# Autodesk Inventor assembly: Factions_Council
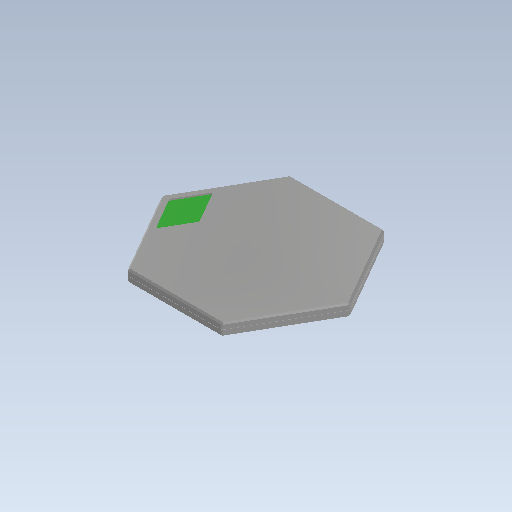
[picture p0: Inventor's stored thumbnail of the model, 512x512]
Saved by Autodesk Inventor 2021 (Build 250183000, 183)
## iProperties
Created: 2023-03-16
Part Number: Factions_Council
Document SubType Name: Assembly
Designer: Bradley
Author: Bradley
## Documents named in this file (7)
- C:\Users\Bradley\Git\TI4\Factions\Factions_Council.iam
- C:\Users\Bradley\Git\TI4\Factions\Factions_Lid.ipt
- C:\Users\Bradley\Git\TI4\Components\FactionSpecial_Council_Cards_All.ipt
- C:\Users\Bradley\Git\TI4\Components\FactionSpecial_Council_ControlMarker_Single.ipt
- C:\Users\Bradley\Git\TI4\Components\FactionSpecial_Council_Home.ipt
- C:\Users\Bradley\Git\TI4\Factions\Factions_BaseCouncil.ipt
- C:\Users\Bradley\Git\TI4\Components\FactionSpecial_Council_CommandToken_Single.ipt
## Components (38 placed, 6 different names)
1. Factions_BaseCouncil:1 — Mate:1, Mate:3, Mate:4, Mate:5, Mate:8, Mate:9, Mate:10, Mate:21, Mate:22, Mate:23, Mate:24, Mate:25, Mate:26, Mate:27, Mate:28, Mate:29, Mate:30, Mate:32, Mate:33, Mate:35, Mate:36, Mate:37, Mate:38, Mate:39, Mate:40, Mate:41, Mate:52, Mate:53, Mate:54, Mate:55, Mate:56, Mate:57, Mate:58, Mate:60, Mate:61, Mate:63, Mate:65, Flush:47, Flush:48
2. Factions_Lid:1 — Mate:1, Flush:47, Flush:48
3. FactionSpecial_Council_Cards_All:1 — Mate:3, Mate:4, Mate:5
4. FactionSpecial_Council_CommandToken_Single:1 — Mate:42, Flush:27, Flush:29, Mate:52, Mate:57, Mate:58, Mate:59
5. FactionSpecial_Council_CommandToken_Single:10
6. FactionSpecial_Council_CommandToken_Single:11 — Mate:55, Mate:63, Mate:64, Mate:66
7. FactionSpecial_Council_CommandToken_Single:12
8. FactionSpecial_Council_CommandToken_Single:13
9. FactionSpecial_Council_CommandToken_Single:14 — Mate:56, Mate:65, Mate:66
10. FactionSpecial_Council_CommandToken_Single:15
11. FactionSpecial_Council_CommandToken_Single:16
12. FactionSpecial_Council_CommandToken_Single:2 — Mate:42, Mate:43, Flush:27, Flush:28, Flush:29, Flush:30
13. FactionSpecial_Council_CommandToken_Single:3 — Mate:43, Flush:28, Flush:30
14. FactionSpecial_Council_CommandToken_Single:4 — Mate:39, Mate:40, Mate:41
15. FactionSpecial_Council_CommandToken_Single:5 — Mate:53, Mate:59, Mate:60, Mate:62
16. FactionSpecial_Council_CommandToken_Single:6
17. FactionSpecial_Council_CommandToken_Single:7
18. FactionSpecial_Council_CommandToken_Single:8 — Mate:54, Mate:61, Mate:62, Mate:64
19. FactionSpecial_Council_CommandToken_Single:9
20. FactionSpecial_Council_ControlMarker_Single:1 — Mate:6, Flush:4, Flush:5, Mate:8, Mate:9, Mate:10
21. FactionSpecial_Council_ControlMarker_Single:10 — Mate:23, Mate:30, Mate:31
22. FactionSpecial_Council_ControlMarker_Single:11
23. FactionSpecial_Council_ControlMarker_Single:12
24. FactionSpecial_Council_ControlMarker_Single:13 — Mate:24, Mate:28, Mate:29, Mate:31
25. FactionSpecial_Council_ControlMarker_Single:14
26. FactionSpecial_Council_ControlMarker_Single:15
27. FactionSpecial_Council_ControlMarker_Single:16 — Mate:25, Mate:26, Mate:27
28. FactionSpecial_Council_ControlMarker_Single:17
29. FactionSpecial_Council_ControlMarker_Single:18
30. FactionSpecial_Council_ControlMarker_Single:2 — Mate:6, Mate:7, Flush:3, Flush:4, Flush:5, Flush:6
31. FactionSpecial_Council_ControlMarker_Single:3 — Mate:7, Flush:3, Flush:6
32. FactionSpecial_Council_ControlMarker_Single:4 — Mate:21, Mate:34, Mate:35
33. FactionSpecial_Council_ControlMarker_Single:5
34. FactionSpecial_Council_ControlMarker_Single:6
35. FactionSpecial_Council_ControlMarker_Single:7 — Mate:22, Mate:32, Mate:33, Mate:34
36. FactionSpecial_Council_ControlMarker_Single:8
37. FactionSpecial_Council_ControlMarker_Single:9
38. FactionSpecial_Council_Home:1 — Mate:36, Mate:37, Mate:38
## Relationships (111: Mate 65, Flush 46)
- Mate:1: Factions_BaseCouncil:1 ↔ Factions_Lid:1
- Mate:3: Factions_BaseCouncil:1 ↔ FactionSpecial_Council_Cards_All:1
- Mate:4 (0.5 mm): Factions_BaseCouncil:1 ↔ FactionSpecial_Council_Cards_All:1
- Mate:5 (0.5 mm): Factions_BaseCouncil:1 ↔ FactionSpecial_Council_Cards_All:1
- Mate:6: FactionSpecial_Council_ControlMarker_Single:1 ↔ FactionSpecial_Council_ControlMarker_Single:2
- Mate:7: FactionSpecial_Council_ControlMarker_Single:2 ↔ FactionSpecial_Council_ControlMarker_Single:3
- Flush:3: FactionSpecial_Council_ControlMarker_Single:2 ↔ FactionSpecial_Council_ControlMarker_Single:3
- Flush:4: FactionSpecial_Council_ControlMarker_Single:1 ↔ FactionSpecial_Council_ControlMarker_Single:2
- Flush:5: FactionSpecial_Council_ControlMarker_Single:1 ↔ FactionSpecial_Council_ControlMarker_Single:2
- Flush:6: FactionSpecial_Council_ControlMarker_Single:2 ↔ FactionSpecial_Council_ControlMarker_Single:3
- Mate:8: Factions_BaseCouncil:1 ↔ FactionSpecial_Council_ControlMarker_Single:1
- Mate:9 (0.5 mm): Factions_BaseCouncil:1 ↔ FactionSpecial_Council_ControlMarker_Single:1
- Mate:10 (0.5 mm): Factions_BaseCouncil:1 ↔ FactionSpecial_Council_ControlMarker_Single:1
- [Mate]: FactionSpecial_Council_ControlMarker_Single:4 ↔ FactionSpecial_Council_ControlMarker_Single:5
- [Mate]: FactionSpecial_Council_ControlMarker_Single:5 ↔ FactionSpecial_Council_ControlMarker_Single:6
- [Flush]: FactionSpecial_Council_ControlMarker_Single:5 ↔ FactionSpecial_Council_ControlMarker_Single:6
- [Flush]: FactionSpecial_Council_ControlMarker_Single:4 ↔ FactionSpecial_Council_ControlMarker_Single:5
- [Flush]: FactionSpecial_Council_ControlMarker_Single:4 ↔ FactionSpecial_Council_ControlMarker_Single:5
- [Flush]: FactionSpecial_Council_ControlMarker_Single:5 ↔ FactionSpecial_Council_ControlMarker_Single:6
- [Mate]: FactionSpecial_Council_ControlMarker_Single:7 ↔ FactionSpecial_Council_ControlMarker_Single:8
- [Mate]: FactionSpecial_Council_ControlMarker_Single:8 ↔ FactionSpecial_Council_ControlMarker_Single:9
- [Flush]: FactionSpecial_Council_ControlMarker_Single:8 ↔ FactionSpecial_Council_ControlMarker_Single:9
- [Flush]: FactionSpecial_Council_ControlMarker_Single:7 ↔ FactionSpecial_Council_ControlMarker_Single:8
- [Flush]: FactionSpecial_Council_ControlMarker_Single:7 ↔ FactionSpecial_Council_ControlMarker_Single:8
- [Flush]: FactionSpecial_Council_ControlMarker_Single:8 ↔ FactionSpecial_Council_ControlMarker_Single:9
- [Mate]: FactionSpecial_Council_ControlMarker_Single:10 ↔ FactionSpecial_Council_ControlMarker_Single:11
- [Mate]: FactionSpecial_Council_ControlMarker_Single:11 ↔ FactionSpecial_Council_ControlMarker_Single:12
- [Flush]: FactionSpecial_Council_ControlMarker_Single:11 ↔ FactionSpecial_Council_ControlMarker_Single:12
- [Flush]: FactionSpecial_Council_ControlMarker_Single:10 ↔ FactionSpecial_Council_ControlMarker_Single:11
- [Flush]: FactionSpecial_Council_ControlMarker_Single:10 ↔ FactionSpecial_Council_ControlMarker_Single:11
- [Flush]: FactionSpecial_Council_ControlMarker_Single:11 ↔ FactionSpecial_Council_ControlMarker_Single:12
- [Mate]: FactionSpecial_Council_ControlMarker_Single:13 ↔ FactionSpecial_Council_ControlMarker_Single:14
- [Mate]: FactionSpecial_Council_ControlMarker_Single:14 ↔ FactionSpecial_Council_ControlMarker_Single:15
- [Flush]: FactionSpecial_Council_ControlMarker_Single:14 ↔ FactionSpecial_Council_ControlMarker_Single:15
- [Flush]: FactionSpecial_Council_ControlMarker_Single:13 ↔ FactionSpecial_Council_ControlMarker_Single:14
- [Flush]: FactionSpecial_Council_ControlMarker_Single:13 ↔ FactionSpecial_Council_ControlMarker_Single:14
- [Flush]: FactionSpecial_Council_ControlMarker_Single:14 ↔ FactionSpecial_Council_ControlMarker_Single:15
- [Mate]: FactionSpecial_Council_ControlMarker_Single:16 ↔ FactionSpecial_Council_ControlMarker_Single:17
- [Mate]: FactionSpecial_Council_ControlMarker_Single:17 ↔ FactionSpecial_Council_ControlMarker_Single:18
- [Flush]: FactionSpecial_Council_ControlMarker_Single:17 ↔ FactionSpecial_Council_ControlMarker_Single:18
- [Flush]: FactionSpecial_Council_ControlMarker_Single:16 ↔ FactionSpecial_Council_ControlMarker_Single:17
- [Flush]: FactionSpecial_Council_ControlMarker_Single:16 ↔ FactionSpecial_Council_ControlMarker_Single:17
- [Flush]: FactionSpecial_Council_ControlMarker_Single:17 ↔ FactionSpecial_Council_ControlMarker_Single:18
- Mate:21: Factions_BaseCouncil:1 ↔ FactionSpecial_Council_ControlMarker_Single:4
- Mate:22: Factions_BaseCouncil:1 ↔ FactionSpecial_Council_ControlMarker_Single:7
- Mate:23: Factions_BaseCouncil:1 ↔ FactionSpecial_Council_ControlMarker_Single:10
- Mate:24: Factions_BaseCouncil:1 ↔ FactionSpecial_Council_ControlMarker_Single:13
- Mate:25: Factions_BaseCouncil:1 ↔ FactionSpecial_Council_ControlMarker_Single:16
- Mate:26 (0.5 mm): Factions_BaseCouncil:1 ↔ FactionSpecial_Council_ControlMarker_Single:16
- Mate:27 (0.5 mm): Factions_BaseCouncil:1 ↔ FactionSpecial_Council_ControlMarker_Single:16
- Mate:28 (0.5 mm): Factions_BaseCouncil:1 ↔ FactionSpecial_Council_ControlMarker_Single:13
- Mate:29 (0.5 mm): Factions_BaseCouncil:1 ↔ FactionSpecial_Council_ControlMarker_Single:13
- Mate:30 (0.5 mm): Factions_BaseCouncil:1 ↔ FactionSpecial_Council_ControlMarker_Single:10
- Mate:31 (0.5 mm): FactionSpecial_Council_ControlMarker_Single:10 ↔ FactionSpecial_Council_ControlMarker_Single:13
- Mate:32 (0.5 mm): Factions_BaseCouncil:1 ↔ FactionSpecial_Council_ControlMarker_Single:7
- Mate:33 (0.5 mm): Factions_BaseCouncil:1 ↔ FactionSpecial_Council_ControlMarker_Single:7
- Mate:34 (0.5 mm): FactionSpecial_Council_ControlMarker_Single:4 ↔ FactionSpecial_Council_ControlMarker_Single:7
- Mate:35 (0.5 mm): Factions_BaseCouncil:1 ↔ FactionSpecial_Council_ControlMarker_Single:4
- Mate:36: Factions_BaseCouncil:1 ↔ FactionSpecial_Council_Home:1
- Mate:37 (0.5 mm): Factions_BaseCouncil:1 ↔ FactionSpecial_Council_Home:1
- Mate:38 (0.5 mm): Factions_BaseCouncil:1 ↔ FactionSpecial_Council_Home:1
- Mate:39: Factions_BaseCouncil:1 ↔ FactionSpecial_Council_CommandToken_Single:4
- Mate:40 (0.5 mm): Factions_BaseCouncil:1 ↔ FactionSpecial_Council_CommandToken_Single:4
- Mate:41 (0.5 mm): Factions_BaseCouncil:1 ↔ FactionSpecial_Council_CommandToken_Single:4
- Mate:42: FactionSpecial_Council_CommandToken_Single:1 ↔ FactionSpecial_Council_CommandToken_Single:2
- Mate:43: FactionSpecial_Council_CommandToken_Single:2 ↔ FactionSpecial_Council_CommandToken_Single:3
- Flush:27: FactionSpecial_Council_CommandToken_Single:1 ↔ FactionSpecial_Council_CommandToken_Single:2
- Flush:28: FactionSpecial_Council_CommandToken_Single:2 ↔ FactionSpecial_Council_CommandToken_Single:3
- Flush:29: FactionSpecial_Council_CommandToken_Single:1 ↔ FactionSpecial_Council_CommandToken_Single:2
- Flush:30: FactionSpecial_Council_CommandToken_Single:2 ↔ FactionSpecial_Council_CommandToken_Single:3
- [Mate]: FactionSpecial_Council_CommandToken_Single:5 ↔ FactionSpecial_Council_CommandToken_Single:6
- [Mate]: FactionSpecial_Council_CommandToken_Single:6 ↔ FactionSpecial_Council_CommandToken_Single:7
- [Flush]: FactionSpecial_Council_CommandToken_Single:5 ↔ FactionSpecial_Council_CommandToken_Single:6
- [Flush]: FactionSpecial_Council_CommandToken_Single:6 ↔ FactionSpecial_Council_CommandToken_Single:7
- [Flush]: FactionSpecial_Council_CommandToken_Single:5 ↔ FactionSpecial_Council_CommandToken_Single:6
- [Flush]: FactionSpecial_Council_CommandToken_Single:6 ↔ FactionSpecial_Council_CommandToken_Single:7
- [Mate]: FactionSpecial_Council_CommandToken_Single:8 ↔ FactionSpecial_Council_CommandToken_Single:9
- [Mate]: FactionSpecial_Council_CommandToken_Single:10 ↔ FactionSpecial_Council_CommandToken_Single:9
- [Flush]: FactionSpecial_Council_CommandToken_Single:8 ↔ FactionSpecial_Council_CommandToken_Single:9
- [Flush]: FactionSpecial_Council_CommandToken_Single:10 ↔ FactionSpecial_Council_CommandToken_Single:9
- [Flush]: FactionSpecial_Council_CommandToken_Single:8 ↔ FactionSpecial_Council_CommandToken_Single:9
- [Flush]: FactionSpecial_Council_CommandToken_Single:10 ↔ FactionSpecial_Council_CommandToken_Single:9
- [Mate]: FactionSpecial_Council_CommandToken_Single:11 ↔ FactionSpecial_Council_CommandToken_Single:12
- [Mate]: FactionSpecial_Council_CommandToken_Single:12 ↔ FactionSpecial_Council_CommandToken_Single:13
- [Flush]: FactionSpecial_Council_CommandToken_Single:11 ↔ FactionSpecial_Council_CommandToken_Single:12
- [Flush]: FactionSpecial_Council_CommandToken_Single:12 ↔ FactionSpecial_Council_CommandToken_Single:13
- [Flush]: FactionSpecial_Council_CommandToken_Single:11 ↔ FactionSpecial_Council_CommandToken_Single:12
- [Flush]: FactionSpecial_Council_CommandToken_Single:12 ↔ FactionSpecial_Council_CommandToken_Single:13
- [Mate]: FactionSpecial_Council_CommandToken_Single:14 ↔ FactionSpecial_Council_CommandToken_Single:15
- [Mate]: FactionSpecial_Council_CommandToken_Single:15 ↔ FactionSpecial_Council_CommandToken_Single:16
- [Flush]: FactionSpecial_Council_CommandToken_Single:14 ↔ FactionSpecial_Council_CommandToken_Single:15
- [Flush]: FactionSpecial_Council_CommandToken_Single:15 ↔ FactionSpecial_Council_CommandToken_Single:16
- [Flush]: FactionSpecial_Council_CommandToken_Single:14 ↔ FactionSpecial_Council_CommandToken_Single:15
- [Flush]: FactionSpecial_Council_CommandToken_Single:15 ↔ FactionSpecial_Council_CommandToken_Single:16
- Mate:52: Factions_BaseCouncil:1 ↔ FactionSpecial_Council_CommandToken_Single:1
- Mate:53: Factions_BaseCouncil:1 ↔ FactionSpecial_Council_CommandToken_Single:5
- Mate:54: Factions_BaseCouncil:1 ↔ FactionSpecial_Council_CommandToken_Single:8
- Mate:55: Factions_BaseCouncil:1 ↔ FactionSpecial_Council_CommandToken_Single:11
- Mate:56: Factions_BaseCouncil:1 ↔ FactionSpecial_Council_CommandToken_Single:14
- Mate:57 (0.5 mm): Factions_BaseCouncil:1 ↔ FactionSpecial_Council_CommandToken_Single:1
- Mate:58 (0.5 mm): Factions_BaseCouncil:1 ↔ FactionSpecial_Council_CommandToken_Single:1
- Mate:59 (0.5 mm): FactionSpecial_Council_CommandToken_Single:1 ↔ FactionSpecial_Council_CommandToken_Single:5
- Mate:60 (0.5 mm): Factions_BaseCouncil:1 ↔ FactionSpecial_Council_CommandToken_Single:5
- Mate:61 (0.5 mm): Factions_BaseCouncil:1 ↔ FactionSpecial_Council_CommandToken_Single:8
- Mate:62 (0.5 mm): FactionSpecial_Council_CommandToken_Single:5 ↔ FactionSpecial_Council_CommandToken_Single:8
- Mate:63 (0.5 mm): Factions_BaseCouncil:1 ↔ FactionSpecial_Council_CommandToken_Single:11
- Mate:64 (0.5 mm): FactionSpecial_Council_CommandToken_Single:11 ↔ FactionSpecial_Council_CommandToken_Single:8
- Mate:65 (0.5 mm): Factions_BaseCouncil:1 ↔ FactionSpecial_Council_CommandToken_Single:14
- Mate:66 (0.5 mm): FactionSpecial_Council_CommandToken_Single:11 ↔ FactionSpecial_Council_CommandToken_Single:14
- Flush:47: Factions_BaseCouncil:1 ↔ Factions_Lid:1
- Flush:48: Factions_BaseCouncil:1 ↔ Factions_Lid:1
## Named parameters: d120_d111 = 0 mm, d121_d112 = 0 mm, d122_d113 = 0 mm, d123_d114 = 0 mm, d124_d115 = 0 mm, d125_d116 = 0 mm, d126_d111 = 0 mm, d127_d112 = 0 mm, d128_d113 = 0 mm, d129_d114 = 0 mm, d130_d115 = 0 mm, d131_d116 = 0 mm, d132_d111 = 0 mm, d133_d112 = 0 mm, d134_d113 = 0 mm, d135_d114 = 0 mm, d136_d115 = 0 mm, d137_d116 = 0 mm, d138_d111 = 0 mm, d139_d112 = 0 mm, d140_d113 = 0 mm, d141_d114 = 0 mm, d142_d115 = 0 mm, d143_d116 = 0 mm, d144_d111 = 0 mm, d145_d112 = 0 mm, d146_d113 = 0 mm, d147_d114 = 0 mm, d148_d115 = 0 mm, d149_d116 = 0 mm, d177_d171 = 0 mm, d178_d172 = 0 mm, d179_d173 = 0 mm, d180_d174 = 0 mm, d181_d175 = 0 mm, d182_d176 = 0 mm, d183_d171 = 0 mm, d184_d172 = 0 mm, d185_d173 = 0 mm, d186_d174 = 0 mm, d187_d175 = 0 mm, d188_d176 = 0 mm, d189_d171 = 0 mm, d190_d172 = 0 mm, d191_d173 = 0 mm, d192_d174 = 0 mm, d193_d175 = 0 mm, d194_d176 = 0 mm, d195_d171 = 0 mm, d196_d172 = 0 mm, d197_d173 = 0 mm, d198_d174 = 0 mm, d199_d175 = 0 mm, d200_d176 = 0 mm
